# Autodesk Inventor assembly: CoreBot
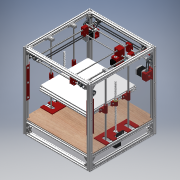
[picture p0: Inventor's stored thumbnail of the model, 180x180]
Saved by Autodesk Inventor 2018 (Build 220112000, 112)
## iProperties
Part Number: CoreBot
Material: Generisch
Document SubType Name: Assembly
Designer: Till
Mass: 5551.29 g
Surface Area: 17511.4 cm^2
Volume: 2427.9 cm^3
Density: 2.28646 g/cm^3
Author: Till
## Documents named in this file (14)
- C:\Users\Till\Dropbox\Ultibox\ultibox\cad\Ultibox.iam
- C:\Users\Till\Dropbox\Ultibox\ultibox\cad\Alu Ramen.iam
- C:\Users\Till\Dropbox\Ultibox\ultibox\cad\Z gantry.iam
- C:\Users\Till\Dropbox\Ultibox\ultibox\cad\UM gantry.iam
- C:\Users\Till\Dropbox\Ultibox\ultibox\cad\Panel.ipt
- C:\Users\Till\Dropbox\Ultibox\ultibox\cad\M3 x 10.ipt
- C:\Users\Till\Dropbox\Ultibox\ultibox\cad\Smoothieboard_X5.ipt
- C:\Users\Till\Dropbox\Ultibox\ultibox\cad\Y-Endstop holder.ipt
- C:\Users\Till\Dropbox\Ultibox\ultibox\cad\X-Endstop holder mount.ipt
- C:\Users\Till\Dropbox\Ultibox\ultibox\cad\Z-Endstop mount.ipt
- C:\Users\Till\Dropbox\Ultibox\ultibox\cad\LED strip mount.ipt
- C:\Users\Till\Dropbox\Ultibox\ultibox\cad\unterlegscheibe_iso_7093-4-140_hv.ipt
- C:\Users\Till\Dropbox\Ultibox\ultibox\cad\screw_iso14580-m4x10-4_8.ipt
- C:\Users\Till\Dropbox\Ultibox\ultibox\cad\X-Endstop holdermount.ipt
## Components (78 placed, 12 different names)
1. aluminium frame [sub-assembly] — Passend:1, Fluchtend:1, Passend:2, Passend:8, Passend:12, Fluchtend:2, Passend:13, Passend:15, Fluchtend:3, Passend:17, Passend:18, Fluchtend:4, Fluchtend:5, Passend:19, Fluchtend:6, Passend:21, Fluchtend:7, Fluchtend:8, Passend:32, Fluchtend:12, Passend:33, Passend:34, Fluchtend:13, Passend:35, Fluchtend:14, Fluchtend:15, Passend:36, Passend:37, Fluchtend:16, Fluchtend:17, Passend:38, Passend:39
2. Z gantry [sub-assembly] — Passend:1, Fluchtend:1, Passend:2
3. XY gantry [sub-assembly] — Passend:12, Fluchtend:2, Passend:13
4. Smoothieboard_X5:1 — Passend:32
5. Y-endstop mount — Fluchtend:12, Passend:33, Passend:34
6. X-endstop  mount — Fluchtend:13, Passend:35, Fluchtend:14
7. Z-endstop mount — Fluchtend:15
8. Panel:1 — Passend:19, Passend:20, Fluchtend:6, Passend:22, Passend:23, Passend:24, Passend:25
9. Panel:2 — Passend:18, Fluchtend:4, Fluchtend:5, Passend:20, Passend:26, Passend:27, Passend:28
10. Panel:3 — Passend:17, Passend:21, Fluchtend:7, Fluchtend:8, Passend:29, Passend:30, Passend:31
11. LED strip mount:1 — Passend:36, Fluchtend:17, Passend:38, Passend:52, Passend:53, Passend:54, Passend:59
12. LED strip mount:2 — Passend:37, Fluchtend:16, Passend:39, Passend:55, Passend:56, Passend:57, Passend:58
13. unterlegscheibe_iso_7093-4-140_hv:1 — Passend:45, Passend:49, Fluchtend:18, Fluchtend:19
14. unterlegscheibe_iso_7093-4-140_hv:2 — Passend:44, Passend:50, Fluchtend:19
15. unterlegscheibe_iso_7093-4-140_hv:3 — Passend:43, Passend:48, Fluchtend:18, Passend:58
16. unterlegscheibe_iso_7093-4-140_hv:4 — Passend:42, Passend:47, Fluchtend:20, Fluchtend:21
17. unterlegscheibe_iso_7093-4-140_hv:5 — Passend:40, Passend:46, Fluchtend:20
18. unterlegscheibe_iso_7093-4-140_hv:6 — Passend:41, Passend:51, Fluchtend:21, Passend:59
19. screw_iso14580-m4x10-4_8:1 — Passend:44, Passend:50, Passend:55
20. screw_iso14580-m4x10-4_8:2 — Passend:45, Passend:49, Passend:56
21. screw_iso14580-m4x10-4_8:3 — Passend:43, Passend:48, Passend:57
22. screw_iso14580-m4x10-4_8:4 — Passend:42, Passend:47, Passend:53
23. screw_iso14580-m4x10-4_8:5 — Passend:41, Passend:51, Passend:52
24. screw_iso14580-m4x10-4_8:6 — Passend:40, Passend:46, Passend:54
25. M3 x 10:54 — Fluchtend:10, Passend:30
26. M3 x 10:56
27. M3 x 10:57
28. M3 x 10:58
29. M3 x 10:59
30. M3 x 10:60
31. M3 x 10:61
32. M3 x 10:62
33. M3 x 10:63
34. M3 x 10:64
35. M3 x 10:55 — Fluchtend:10, Passend:29, Passend:31
36. M3 x 10:65
37. M3 x 10:66
38. M3 x 10:67
39. M3 x 10:68
40. M3 x 10:69
41. M3 x 10:70
42. M3 x 10:71
43. M3 x 10:37 — Fluchtend:9, Passend:27
44. M3 x 10:38
45. M3 x 10:39
46. M3 x 10:40
47. M3 x 10:41
48. M3 x 10:42
49. M3 x 10:43
50. M3 x 10:44
51. M3 x 10:45
52. M3 x 10:46
53. M3 x 10:36 — Fluchtend:9, Passend:26, Passend:28
54. M3 x 10:47
55. M3 x 10:48
56. M3 x 10:49
57. M3 x 10:50
58. M3 x 10:51
59. M3 x 10:52
60. M3 x 10:53
61. M3 x 10:18 — Passend:22, Passend:23
62. M3 x 10:19
63. M3 x 10:20
64. M3 x 10:21
65. M3 x 10:22
66. M3 x 10:23
67. M3 x 10:24
68. M3 x 10:25
69. M3 x 10:26
70. M3 x 10:27
71. M3 x 10:28 — Passend:24, Passend:25
72. M3 x 10:29
73. M3 x 10:30
74. M3 x 10:31
75. M3 x 10:32
76. M3 x 10:33
77. M3 x 10:34
78. M3 x 10:35
## Component patterns: right panel horizontal (10 elements), right panel vertical (8 elements), left panel horizontal (10 elements), left panel vertical (8 elements), back panel horizontal (10 elements), back panel vertical (8 elements)
## Relationships (69: Mate 49, Flush 20)
- Passend:1 [Mate]: aluminium frame ↔ Z gantry
- Fluchtend:1 [Flush] (3 mm): aluminium frame ↔ Z gantry
- Passend:2 [Mate] (115 mm): aluminium frame ↔ Z gantry
- Passend:8 [Mate]: aluminium frame
- Passend:12 [Mate]: aluminium frame ↔ XY gantry
- Fluchtend:2 [Flush] (3.5 mm): aluminium frame ↔ XY gantry
- Passend:13 [Mate] (0.1 mm): aluminium frame ↔ XY gantry
- Passend:15 [Mate]: aluminium frame
- Fluchtend:3 [Flush]: aluminium frame
- Passend:17 [Mate]: aluminium frame ↔ Panel:3
- Passend:18 [Mate]: aluminium frame ↔ Panel:2
- Fluchtend:4 [Flush]: aluminium frame ↔ Panel:2
- Fluchtend:5 [Flush]: aluminium frame ↔ Panel:2
- Passend:19 [Mate]: aluminium frame ↔ Panel:1
- Passend:20 [Mate]: Panel:1 ↔ Panel:2
- Fluchtend:6 [Flush]: aluminium frame ↔ Panel:1
- Passend:21 [Mate]: aluminium frame ↔ Panel:3
- Fluchtend:7 [Flush]: aluminium frame ↔ Panel:3
- Fluchtend:8 [Flush]: aluminium frame ↔ Panel:3
- Passend:22 [Mate]: Panel:1 ↔ M3 x 10:18
- Passend:23 [Mate]: Panel:1 ↔ M3 x 10:18
- Passend:24 [Mate]: Panel:1 ↔ M3 x 10:28
- Passend:25 [Mate]: Panel:1 ↔ M3 x 10:28
- Fluchtend:9 [Flush]: M3 x 10:37 ↔ M3 x 10:36
- Passend:26 [Mate]: Panel:2 ↔ M3 x 10:36
- Passend:27 [Mate]: Panel:2 ↔ M3 x 10:37
- Passend:28 [Mate]: Panel:2 ↔ M3 x 10:36
- Fluchtend:10 [Flush]: M3 x 10:54 ↔ M3 x 10:55
- Passend:29 [Mate]: Panel:3 ↔ M3 x 10:55
- Passend:30 [Mate]: Panel:3 ↔ M3 x 10:54
- Passend:31 [Mate]: Panel:3 ↔ M3 x 10:55
- Passend:32 [Mate]: aluminium frame ↔ Smoothieboard_X5:1
- Fluchtend:12 [Flush]: aluminium frame ↔ Y-endstop mount
- Passend:33 [Mate]: aluminium frame ↔ Y-endstop mount
- Passend:34 [Mate]: aluminium frame ↔ Y-endstop mount
- Fluchtend:13 [Flush]: aluminium frame ↔ X-endstop  mount
- Passend:35 [Mate]: aluminium frame ↔ X-endstop  mount
- Fluchtend:14 [Flush]: aluminium frame ↔ X-endstop  mount
- Fluchtend:15 [Flush]: aluminium frame ↔ Z-endstop mount
- Passend:36 [Mate]: aluminium frame ↔ LED strip mount:1
- Passend:37 [Mate]: aluminium frame ↔ LED strip mount:2
- Fluchtend:16 [Flush]: aluminium frame ↔ LED strip mount:2
- Fluchtend:17 [Flush]: aluminium frame ↔ LED strip mount:1
- Passend:38 [Mate] (60 mm): aluminium frame ↔ LED strip mount:1
- Passend:39 [Mate] (60 mm): aluminium frame ↔ LED strip mount:2
- Passend:40 [Mate]: unterlegscheibe_iso_7093-4-140_hv:5 ↔ screw_iso14580-m4x10-4_8:6
- Passend:41 [Mate]: unterlegscheibe_iso_7093-4-140_hv:6 ↔ screw_iso14580-m4x10-4_8:5
- Passend:42 [Mate]: unterlegscheibe_iso_7093-4-140_hv:4 ↔ screw_iso14580-m4x10-4_8:4
- Passend:43 [Mate]: unterlegscheibe_iso_7093-4-140_hv:3 ↔ screw_iso14580-m4x10-4_8:3
- Passend:44 [Mate]: unterlegscheibe_iso_7093-4-140_hv:2 ↔ screw_iso14580-m4x10-4_8:1
- Passend:45 [Mate]: unterlegscheibe_iso_7093-4-140_hv:1 ↔ screw_iso14580-m4x10-4_8:2
- Passend:46 [Mate]: unterlegscheibe_iso_7093-4-140_hv:5 ↔ screw_iso14580-m4x10-4_8:6
- Passend:47 [Mate]: unterlegscheibe_iso_7093-4-140_hv:4 ↔ screw_iso14580-m4x10-4_8:4
- Passend:48 [Mate]: unterlegscheibe_iso_7093-4-140_hv:3 ↔ screw_iso14580-m4x10-4_8:3
- Passend:49 [Mate]: unterlegscheibe_iso_7093-4-140_hv:1 ↔ screw_iso14580-m4x10-4_8:2
- Passend:50 [Mate]: unterlegscheibe_iso_7093-4-140_hv:2 ↔ screw_iso14580-m4x10-4_8:1
- Passend:51 [Mate]: unterlegscheibe_iso_7093-4-140_hv:6 ↔ screw_iso14580-m4x10-4_8:5
- Passend:52 [Mate]: LED strip mount:1 ↔ screw_iso14580-m4x10-4_8:5
- Passend:53 [Mate]: LED strip mount:1 ↔ screw_iso14580-m4x10-4_8:4
- Passend:54 [Mate]: LED strip mount:1 ↔ screw_iso14580-m4x10-4_8:6
- Fluchtend:18 [Flush]: unterlegscheibe_iso_7093-4-140_hv:1 ↔ unterlegscheibe_iso_7093-4-140_hv:3
- Fluchtend:19 [Flush]: unterlegscheibe_iso_7093-4-140_hv:1 ↔ unterlegscheibe_iso_7093-4-140_hv:2
- Passend:55 [Mate]: LED strip mount:2 ↔ screw_iso14580-m4x10-4_8:1
- Passend:56 [Mate]: LED strip mount:2 ↔ screw_iso14580-m4x10-4_8:2
- Passend:57 [Mate]: LED strip mount:2 ↔ screw_iso14580-m4x10-4_8:3
- Passend:58 [Mate]: LED strip mount:2 ↔ unterlegscheibe_iso_7093-4-140_hv:3
- Fluchtend:20 [Flush]: unterlegscheibe_iso_7093-4-140_hv:4 ↔ unterlegscheibe_iso_7093-4-140_hv:5
- Fluchtend:21 [Flush]: unterlegscheibe_iso_7093-4-140_hv:4 ↔ unterlegscheibe_iso_7093-4-140_hv:6
- Passend:59 [Mate]: LED strip mount:1 ↔ unterlegscheibe_iso_7093-4-140_hv:6
